# Autodesk Inventor assembly: Assembly1
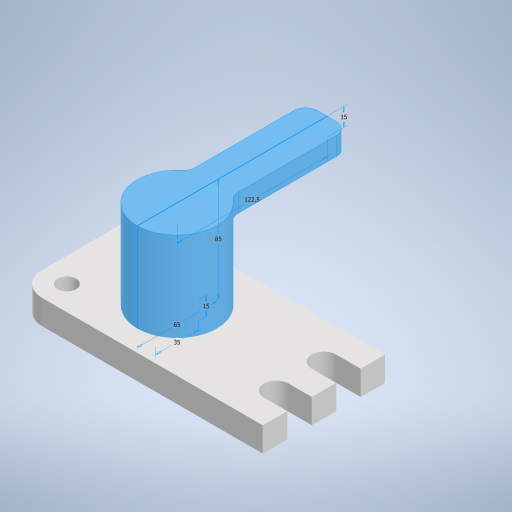
[picture p0: Inventor's stored thumbnail of the model, 512x512]
Saved by Autodesk Inventor 2023 (Build 270158000, 158)
## iProperties
Created: 2023-03-01
Part Number: Assembly1
Document SubType Name: Assembly
Designer: accam
Author: accam
## Documents named in this file (3)
- C:\Users\accam\Documents\Assembly1.iam
- C:\Users\accam\Documents\Wkp 01.03.1.ipt
- C:\Users\accam\Documents\Wkp 01.03.2.ipt
## Components (2 placed, 2 different names)
1. Wkp 01.03.1:2 — Rotational:1
2. Wkp 01.03.2:1 — Rotational:1
## Relationships (1: RevoluteJoint 1)
- Rotational:1 [RevoluteJoint]: Wkp 01.03.1:2 ↔ Wkp 01.03.2:1
